# Autodesk Inventor assembly: shaft support
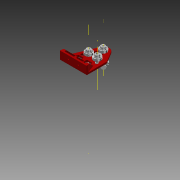
[picture p0: Inventor's stored thumbnail of the model, 180x180]
Saved by Autodesk Inventor 2013 (Build 170138000, 138)
## iProperties
Created: 2015-04-05
Part Number: shaft support
Document SubType Name: Assembly
Designer: Nico
Author: Nico
## Documents named in this file (6)
- D:\Documents\Inventor\Fish Rod laquer Machine\shaft support.iam
- D:\Documents\Inventor\Fish Rod laquer Machine\Rod end holder.ipt
- D:\Documents\Inventor\Fish Rod laquer Machine\608ZZ bearing.ipt
- D:\Documents\Inventor\Content Center Files\R2013\en-US\ISO 7092\ISO 7092 - ST 8 - 140 HV.ipt
- D:\Documents\Inventor\Content Center Files\R2013\en-US\DIN 7984\DIN 7984 - M8 x 25.ipt
- D:\Documents\Inventor\Content Center Files\R2013\en-US\DIN 315\DIN 315 - M8.ipt
## Components (19 placed, 5 different names)
1. Rod end holder:1 — Mate:20, Mate:21, Mate:29, Mate:30, Mate:40, Mate:41
2. 608ZZ bearing:1 — Mate:16, Mate:18, Mate:32
3. 608ZZ bearing:2 — Mate:37, Mate:38, Mate:39
4. 608ZZ bearing:3 — Mate:25, Mate:26, Mate:28
5. DIN 7984 M8 x 25:1 — Mate:1, Mate:22, Mate:23, Mate:24, Mate:25, Mate:27, Mate:47
6. DIN 7984 M8 x 25:2 — Mate:2, Mate:33, Mate:34, Mate:35, Mate:45, Mate:51
7. DIN 7984 M8 x 25:3 — Mate:3, Mate:13, Mate:14, Mate:15, Mate:31
8. ISO 7092 ST 8 - 140 HV:1 — Mate:10, Mate:18, Mate:31
9. ISO 7092 ST 8 - 140 HV:2 — Mate:7, Mate:26, Mate:27
10. ISO 7092 ST 8 - 140 HV:3 — Mate:4, Mate:28, Mate:29
11. ISO 7092 ST 8 - 140 HV:4 — Mate:5, Mate:30, Mate:48
12. ISO 7092 ST 8 - 140 HV:5 — Mate:6, Mate:39, Mate:51
13. ISO 7092 ST 8 - 140 HV:6 — Mate:8, Mate:38, Mate:40
14. ISO 7092 ST 8 - 140 HV:7 — Mate:11, Mate:20, Mate:32
15. ISO 7092 ST 8 - 140 HV:8 — Mate:12, Mate:21, Mate:49
16. ISO 7092 ST 8 - 140 HV:9 — Mate:9, Mate:41, Mate:50
17. DIN 315 M8:1 — Mate:44, Mate:48
18. DIN 315 M8:2 — Mate:43, Mate:49
19. DIN 315 M8:3 — Mate:42, Mate:50
## Relationships (48: Mate 48)
- Mate:1: DIN 7984 M8 x 25:1
- Mate:2: DIN 7984 M8 x 25:2
- Mate:3: DIN 7984 M8 x 25:3
- Mate:4: ISO 7092 ST 8 - 140 HV:3
- Mate:5: ISO 7092 ST 8 - 140 HV:4
- Mate:6: ISO 7092 ST 8 - 140 HV:5
- Mate:7: ISO 7092 ST 8 - 140 HV:2
- Mate:8: ISO 7092 ST 8 - 140 HV:6
- Mate:9: ISO 7092 ST 8 - 140 HV:9
- Mate:10: ISO 7092 ST 8 - 140 HV:1
- Mate:11: ISO 7092 ST 8 - 140 HV:7
- Mate:12: ISO 7092 ST 8 - 140 HV:8
- Mate:13: DIN 7984 M8 x 25:3
- Mate:14: DIN 7984 M8 x 25:3
- Mate:15: DIN 7984 M8 x 25:3
- Mate:16: 608ZZ bearing:1
- Mate:18: 608ZZ bearing:1 ↔ ISO 7092 ST 8 - 140 HV:1
- Mate:20: Rod end holder:1 ↔ ISO 7092 ST 8 - 140 HV:7
- Mate:21: Rod end holder:1 ↔ ISO 7092 ST 8 - 140 HV:8
- Mate:22: DIN 7984 M8 x 25:1
- Mate:23: DIN 7984 M8 x 25:1
- Mate:24: DIN 7984 M8 x 25:1
- Mate:25: 608ZZ bearing:3 ↔ DIN 7984 M8 x 25:1
- Mate:26: 608ZZ bearing:3 ↔ ISO 7092 ST 8 - 140 HV:2
- Mate:27: DIN 7984 M8 x 25:1 ↔ ISO 7092 ST 8 - 140 HV:2
- Mate:28: 608ZZ bearing:3 ↔ ISO 7092 ST 8 - 140 HV:3
- Mate:29: Rod end holder:1 ↔ ISO 7092 ST 8 - 140 HV:3
- Mate:30: Rod end holder:1 ↔ ISO 7092 ST 8 - 140 HV:4
- Mate:31: DIN 7984 M8 x 25:3 ↔ ISO 7092 ST 8 - 140 HV:1
- Mate:32: 608ZZ bearing:1 ↔ ISO 7092 ST 8 - 140 HV:7
- Mate:33: DIN 7984 M8 x 25:2
- Mate:34: DIN 7984 M8 x 25:2
- Mate:35: DIN 7984 M8 x 25:2
- Mate:37: 608ZZ bearing:2
- Mate:38: 608ZZ bearing:2 ↔ ISO 7092 ST 8 - 140 HV:6
- Mate:39: 608ZZ bearing:2 ↔ ISO 7092 ST 8 - 140 HV:5
- Mate:40: Rod end holder:1 ↔ ISO 7092 ST 8 - 140 HV:6
- Mate:41: Rod end holder:1 ↔ ISO 7092 ST 8 - 140 HV:9
- Mate:42: DIN 315 M8:3
- Mate:43: DIN 315 M8:2
- Mate:44: DIN 315 M8:1
- Mate:45: DIN 7984 M8 x 25:2
- Mate:46
- Mate:47: DIN 7984 M8 x 25:1
- Mate:48: ISO 7092 ST 8 - 140 HV:4 ↔ DIN 315 M8:1
- Mate:49: ISO 7092 ST 8 - 140 HV:8 ↔ DIN 315 M8:2
- Mate:50: ISO 7092 ST 8 - 140 HV:9 ↔ DIN 315 M8:3
- Mate:51: DIN 7984 M8 x 25:2 ↔ ISO 7092 ST 8 - 140 HV:5
